# Autodesk Inventor assembly: topstage
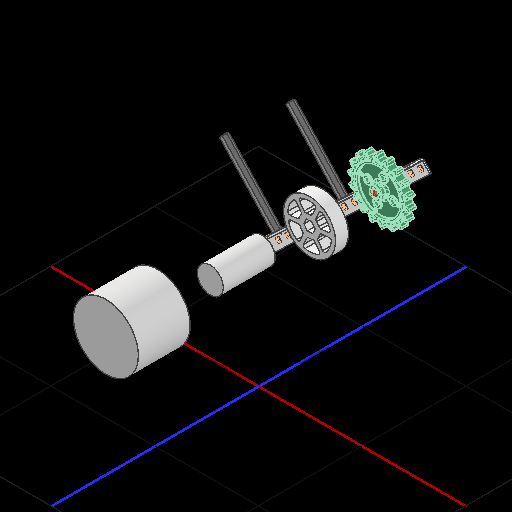
[picture p0: Inventor's stored thumbnail of the model, 512x512]
Saved by Autodesk Inventor 2025.2 (Build 292293000, 293)
## iProperties
Created: 2025-11-17
Part Number: topstage
Document SubType Name: Assembly
Designer: cloudy
Author: cloudy
## Documents named in this file (10)
- C:\Users\cloudy\Documents\AURA_CAD\15\topstage.iam
- C:\Users\cloudy\Documents\AURA_CAD\!lib\Structure\C Channel\Aluminum 1x3x1 Half\Alu C Half 1x3x1x20.ipt
- C:\Users\cloudy\Documents\AURA_CAD\!lib\Motion\Sprockets\9P Sprocket\9P 18T Sprocket, Circle.iam
- C:\Users\cloudy\Documents\AURA_CAD\!lib\Motion\Sprockets\9P Sprocket.iam
- C:\Users\cloudy\Documents\AURA_CAD\15\2.5in roller.ipt
- C:\Users\cloudy\Documents\AURA_CAD\!lib\Structure\Standoff\Standoff 3.00.ipt
- C:\Users\cloudy\Documents\AURA_CAD\!lib\Structure\Standoff.ipt
- C:\Users\cloudy\Documents\AURA_CAD\!lib\Motion\Wheels\Flex Wheels\2.000 Flex Wheel\2.000 30A .500.ipt
- C:\Users\cloudy\Documents\AURA_CAD\!lib\Motion\Wheels\Flex Wheels\2.000 Flex Wheel.ipt
- C:\Users\cloudy\Documents\AURA_CAD\15\1 in roller.ipt
## Components (7 placed, 6 different names)
1. Alu C Half 1x3x1x20:1
2. 9P 18T Sprocket, Circle:1 [sub-assembly]
3. 2.5in roller:1
4. Standoff 3.00:1
5. Standoff 3.00:2
6. 2.000 30A .500:1
7. 1 in roller:1
## Relationships (6: Insert 5, Mate 1)
- [Insert] (12.7 mm): Alu C Half 1x3x1x20:1 ↔ 9P 18T Sprocket, Circle:1
- [Mate]: Alu C Half 1x3x1x20:1 ↔ 2.5in roller:1
- [Insert]: Alu C Half 1x3x1x20:1 ↔ Standoff 3.00:1
- [Insert]: Alu C Half 1x3x1x20:1 ↔ Standoff 3.00:2
- [Insert] (12.7 mm): Alu C Half 1x3x1x20:1 ↔ 2.000 30A .500:1
- [Insert] (25.4 mm): Alu C Half 1x3x1x20:1 ↔ 1 in roller:1
